# Autodesk Inventor assembly: Endstop10mm
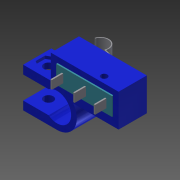
[picture p0: Inventor's stored thumbnail of the model, 180x180]
Saved by Autodesk Inventor 2014 SP1 (Build 180222100, 222)
## iProperties
Created: 2014-03-02
Part Number: Endstop10mm
Document SubType Name: Assembly
Designer: Jack
Author: Jack
## Documents named in this file (3)
- C:\Users\Jack\Sync\MendelMax1.5\InventorParts\Electronics\Endstop10mm.iam
- C:\Users\Jack\Sync\MendelMax1.5\InventorParts\Electronics\EndStopClip10mm.ipt
- C:\Users\Jack\Sync\MendelMax1.5\InventorParts\Electronics\EndStopSwitch.ipt
## Components (2 placed, 2 different names)
1. EndStopClip10mm:1 — Mate:1, Mate:2, Flush:1
2. EndStopSwitch:1 — Mate:1, Mate:2, Flush:1
## Relationships (3: Mate 2, Flush 1)
- Mate:1: EndStopClip10mm:1 ↔ EndStopSwitch:1
- Mate:2: EndStopClip10mm:1 ↔ EndStopSwitch:1
- Flush:1: EndStopClip10mm:1 ↔ EndStopSwitch:1
